# Autodesk Inventor assembly: 6P Sprocket
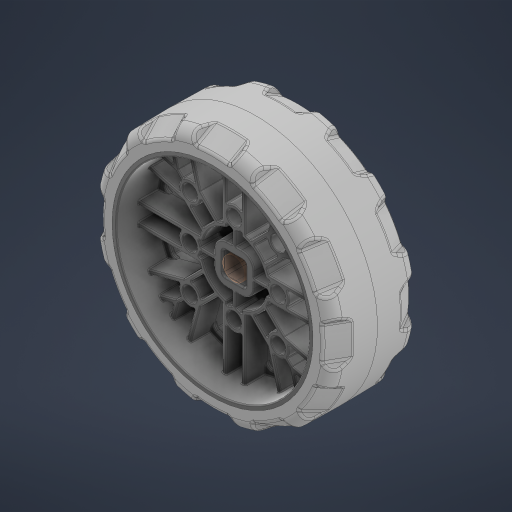
[picture p0: Inventor's stored thumbnail of the model, 512x512]
Saved by Autodesk Inventor 2024 (Build 280153000, 153)
## iProperties
Created: 2022-08-02
Part Number: 6P Sprocket
Document SubType Name: Assembly
Designer: ylu12
Author: ylu12
## Documents named in this file (3)
- D:\vex_robotics\hardware\cad\VEX-CAD-Inventor-1.41\Motion\Wheels\Traction Wheel\2.75 Traction AS, No Insert.iam
- D:\vex_robotics\hardware\cad\VEX-CAD-Inventor-1.41\Motion\Wheels\Reference Files\2.75 Traction Antistatic.ipt
- D:\vex_robotics\hardware\cad\VEX-CAD-Inventor-1.41\Motion\Wheels\Traction Wheel.iam
## Components (1 placed, 1 different names)
1. 2.75 Traction Antistatic:1 — Mate:17, Mate:18, Mate:19
## Relationships (3: Mate 3)
- Mate:17: 2.75 Traction Antistatic:1
- Mate:18: 2.75 Traction Antistatic:1
- Mate:19: 2.75 Traction Antistatic:1
## Named parameters: Thickness = 8.255 mm
